# Autodesk Inventor assembly: USB-1SP16T-83H
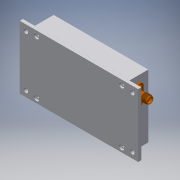
[picture p0: Inventor's stored thumbnail of the model, 180x180]
Saved by Autodesk Inventor 2018 (Build 220112000, 112)
## iProperties
Created: 2019-09-24
Part Number: USB-1SP16T-83H
Document SubType Name: Assembly
Designer: alexanderpollak
Author: alexanderpollak
## Documents named in this file (6)
- C:\Users\alexanderpollak\ownCloud\Inventor\ATA_2019\ATA_RFS_Rack_2019\Parts\RUDAT-6000-30\RUDAT-6000-30.iam
- C:\Users\alexanderpollak\ownCloud\Inventor\ATA_2019\ATA_RFS_Rack_2019\Parts\RUDAT-6000-30\RUDAT-6000-30.ipt
- C:\Users\alexanderpollak\ownCloud\Inventor\ATA_2019\ATA_RFS_Rack_2019\Parts\RUDAT-6000-30\2waysma.ipt
- C:\Users\alexanderpollak\ownCloud\Inventor\ATA_2019\ATA_RFS_Rack_2019\Parts\RUDAT-6000-30\1653983_205161-1.ipt
- C:\Users\alexanderpollak\ownCloud\Inventor\ATA_2019\ATA_RFS_Rack_2019\Parts\RUDAT-6000-30\2342993-1.ipt
- C:\Users\alexanderpollak\ownCloud\Inventor\ATA_2019\ATA_RFS_Rack_2019\Parts\RUDAT-6000-30\RUDAT-6000-30-Bracket.ipt
## Components (6 placed, 5 different names)
1. RUDAT-6000-30:1 — Flush:1, Mate:1, Flush:2, Flush:3, Flush:4, Flush:5, Insert:1, Insert:2, Insert:3, Insert:4
2. 2waysma:4 — Insert:2
3. 2waysma:11 — Insert:1
4. 1653983_205161-1:1 — Flush:1, Mate:1, Flush:2
5. 2342993-1:1 — Flush:3, Flush:4, Flush:5
6. RUDAT-6000-30-Bracket:1 — Insert:3, Insert:4
## Relationships (10: Flush 5, Insert 4, Mate 1)
- Flush:1 (35 mm): RUDAT-6000-30:1 ↔ 1653983_205161-1:1
- Mate:1: RUDAT-6000-30:1 ↔ 1653983_205161-1:1
- Flush:2 (1 mm): RUDAT-6000-30:1 ↔ 1653983_205161-1:1
- Flush:3 (-1 mm): RUDAT-6000-30:1 ↔ 2342993-1:1
- Flush:4 (55 mm): RUDAT-6000-30:1 ↔ 2342993-1:1
- Flush:5 (8 mm): RUDAT-6000-30:1 ↔ 2342993-1:1
- Insert:1: RUDAT-6000-30:1 ↔ 2waysma:11
- Insert:2: RUDAT-6000-30:1 ↔ 2waysma:4
- Insert:3: RUDAT-6000-30:1 ↔ RUDAT-6000-30-Bracket:1
- Insert:4: RUDAT-6000-30:1 ↔ RUDAT-6000-30-Bracket:1
